# Autodesk Inventor assembly: Mesh Assembly
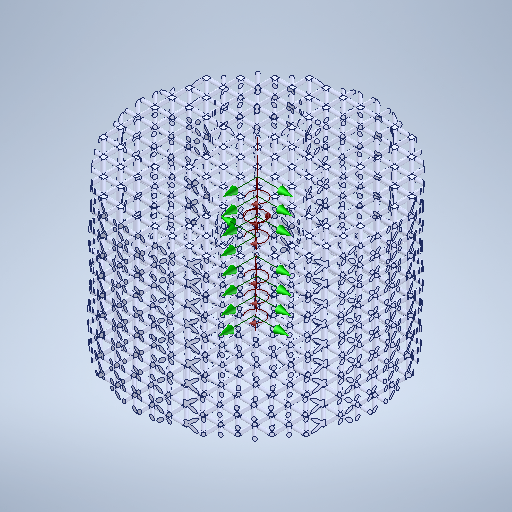
[picture p0: Inventor's stored thumbnail of the model, 512x512]
Saved by Autodesk Inventor 2026.2 (Build 302298000, 298)
## iProperties
Created: 2026-01-18
Part Number: Mesh Assembly
Document SubType Name: Assembly
Designer: daryu
Author: daryu
## Documents named in this file (2)
- C:\Users\daryu\Documents\RE entry capsule\Mesh Assembly.iam
- C:\Users\daryu\Downloads\Lattice.ipt
## Components (9 placed, 1 different names)
1. Lattice:1 — Mate:1, Angle:1, Angle:2, Angle:3
2. Lattice:2 — Mate:1, Mate:2, Angle:1, Angle:2, Angle:3
3. Lattice:3 — Mate:2, Mate:3
4. Lattice:4 — Mate:3, Mate:4
5. Lattice:5 — Mate:4, Mate:5
6. Lattice:6 — Mate:5, Mate:6
7. Lattice:7 — Mate:6, Mate:7
8. Lattice:8 — Mate:7, Mate:8
9. Lattice:9 — Mate:8
## Relationships (11: Mate 8, Angle 3)
- Mate:1: Lattice:1 ↔ Lattice:2
- Mate:2: Lattice:2 ↔ Lattice:3
- Mate:3: Lattice:3 ↔ Lattice:4
- Mate:4: Lattice:4 ↔ Lattice:5
- Angle:1 (0 deg): Lattice:1 ↔ Lattice:2
- Angle:2 (0 deg): Lattice:1 ↔ Lattice:2
- Angle:3 (0 deg): Lattice:1 ↔ Lattice:2
- Mate:5: Lattice:5 ↔ Lattice:6
- Mate:6: Lattice:6 ↔ Lattice:7
- Mate:7: Lattice:7 ↔ Lattice:8
- Mate:8: Lattice:8 ↔ Lattice:9
